# Autodesk Inventor assembly: Assembly1
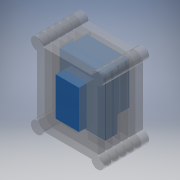
[picture p0: Inventor's stored thumbnail of the model, 180x180]
Saved by Autodesk Inventor 2016 (Build 200138000, 138)
## iProperties
Created: 2017-05-08
Part Number: Assembly1
Document SubType Name: Assembly
Designer: rdiaz
Author: rdiaz
## Documents named in this file (5)
- C:\Users\rdiaz\Desktop\Oled_Optical\Empaque\Assembly1.iam
- C:\Users\rdiaz\Desktop\Oled_Optical\Empaque\Cubiertasensor.ipt
- C:\Users\rdiaz\Desktop\Oled_Optical\Empaque\Modulo.ipt
- C:\Users\rdiaz\Desktop\Oled_Optical\Empaque\cubierta tarjeta.ipt
- C:\Users\rdiaz\Desktop\Oled_Optical\Empaque\cubierta OLED.ipt
## Components (7 placed, 4 different names)
1. Cubiertasensor:3 — Mate:14, Mate:15, Mate:16, Mate:17, Flush:7, Flush:8, Mate:18, Mate:19, Flush:15, Flush:16
2. Modulo:1 — Mate:14, Mate:15, Mate:16
3. Cubiertasensor:4 — Mate:17, Flush:7, Flush:8
4. cubierta tarjeta:1 — Mate:18, Mate:19, Mate:20, Flush:11, Flush:15, Flush:16, Flush:17
5. cubierta tarjeta:2 — Mate:20, Flush:11, Flush:13, Mate:21, Flush:14, Flush:17
6. cubierta OLED:1 — Flush:13, Mate:21, Flush:14, Mate:22, Flush:18, Flush:19
7. cubierta OLED:2 — Mate:22, Flush:18, Flush:19
## Relationships (19: Flush 10, Mate 9)
- Mate:14: Cubiertasensor:3 ↔ Modulo:1
- Mate:15: Cubiertasensor:3 ↔ Modulo:1
- Mate:16: Cubiertasensor:3 ↔ Modulo:1
- Mate:17: Cubiertasensor:3 ↔ Cubiertasensor:4
- Flush:7: Cubiertasensor:3 ↔ Cubiertasensor:4
- Flush:8: Cubiertasensor:3 ↔ Cubiertasensor:4
- Mate:18: Cubiertasensor:3 ↔ cubierta tarjeta:1
- Mate:19: Cubiertasensor:3 ↔ cubierta tarjeta:1
- Mate:20: cubierta tarjeta:1 ↔ cubierta tarjeta:2
- Flush:11: cubierta tarjeta:1 ↔ cubierta tarjeta:2
- Flush:13: cubierta tarjeta:2 ↔ cubierta OLED:1
- Mate:21: cubierta tarjeta:2 ↔ cubierta OLED:1
- Flush:14: cubierta tarjeta:2 ↔ cubierta OLED:1
- Flush:15: Cubiertasensor:3 ↔ cubierta tarjeta:1
- Flush:16: Cubiertasensor:3 ↔ cubierta tarjeta:1
- Flush:17: cubierta tarjeta:1 ↔ cubierta tarjeta:2
- Mate:22: cubierta OLED:1 ↔ cubierta OLED:2
- Flush:18: cubierta OLED:1 ↔ cubierta OLED:2
- Flush:19: cubierta OLED:1 ↔ cubierta OLED:2
